# Autodesk Inventor assembly: 新款四方轴套
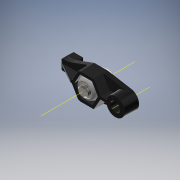
[picture p0: Inventor's stored thumbnail of the model, 180x180]
Saved by Autodesk Inventor 2019.4 (Build 234330000, 330)
## iProperties
Created: 2019-05-20
Part Number: 新款四方轴套
Material: 常规
Document SubType Name: Assembly
Designer: aresp
Author: aresp
## Documents named in this file (4)
- D:\2019-2020TowerTakeOverCad\ncrCadLib\新款四方轴套.iam
- D:\2019-2020TowerTakeOverCad\ncrCadLib\轴相关\细轴新款四方轴承.ipt
- D:\2019-2020TowerTakeOverCad\ncrCadLib\螺丝螺帽\Screw 8-32 x 0.375'' 二号.ipt
- D:\2019-2020TowerTakeOverCad\ncrCadLib\螺丝螺帽\防滑螺帽.ipt
## Components (3 placed, 3 different names)
1. 细轴新款四方轴承:1 — 配合:1, 配合:2, 配合:3, 配合:4
2. Screw 8-32 x 0.375'' 二号:1 — 配合:3, 配合:4
3. 防滑螺帽:1 — 配合:1, 配合:2
## Relationships (4: Mate 4)
- 配合:1 [Mate]: 细轴新款四方轴承:1 ↔ 防滑螺帽:1
- 配合:2 [Mate]: 细轴新款四方轴承:1 ↔ 防滑螺帽:1
- 配合:3 [Mate]: 细轴新款四方轴承:1 ↔ Screw 8-32 x 0.375'' 二号:1
- 配合:4 [Mate] (1.575 mm): 细轴新款四方轴承:1 ↔ Screw 8-32 x 0.375'' 二号:1
